# Autodesk Inventor assembly: Omnibot_battery_module.brd
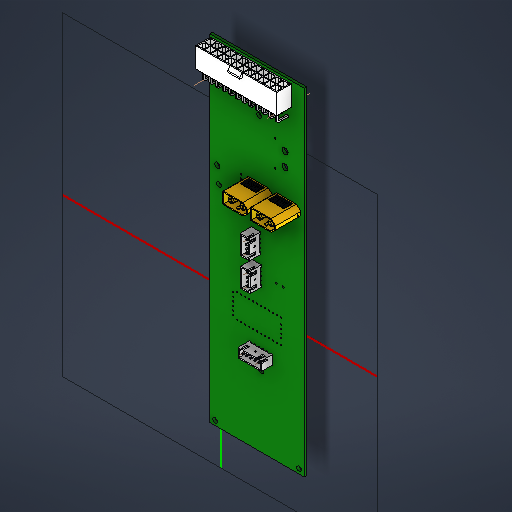
[picture p0: Inventor's stored thumbnail of the model, 512x512]
Saved by Autodesk Inventor 2025 (Build 290162000, 162)
## iProperties
Created: 2024-08-13
Part Number: Omnibot_battery_module.brd
Document SubType Name: Assembly
Designer: IvanPetrov
Author: IvanPetrov
## Documents named in this file (6)
- D:\Projects\OmniBot\design\000.007 - Монитор заряда АКБ.iam
- D:\Projects\OmniBot\design\standart_components\ATX Connector 24pin 90deg\ATX Connector 24pin 90deg.ipt
- D:\Projects\OmniBot\design\standart_components\XT60FemaleConnector.ipt
- D:\Projects\OmniBot\design\standart_components\connectrs\JST - XH - Thru (V) - 4Pin - 2.54mm.ipt
- D:\Projects\OmniBot\design\standart_components\connectrs\JST - XH - Thru (V) - 5Pin - 2.54mm.ipt
- D:\Projects\OmniBot\design\000.007.001 - Плата.ipt
## Components (7 placed, 5 different names)
1. 000.007.001 - Плата:3
2. ATX Connector 24pin 90deg:1 — Угол:5
3. XT60FemaleConnector:1 — Угол:3, Угол:5, Угол:6
4. XT60FemaleConnector:2 — Угол:3, Угол:6
5. JST - XH - Thru (V) - 4Pin - 2.54mm:1
6. JST - XH - Thru (V) - 4Pin - 2.54mm:2
7. JST - XH - Thru (V) - 5Pin - 2.54mm:1
## Relationships (19: Mate 15, Angle 4)
- Угол:3 [Angle] (0 deg): XT60FemaleConnector:1 ↔ XT60FemaleConnector:2
- [Mate]: 000.007.001 - Плата:3 ↔ ATX Connector 24pin 90deg:1
- [Mate]: 000.007.001 - Плата:3 ↔ ATX Connector 24pin 90deg:1
- [Angle] (0 deg): 000.007.001 - Плата:3 ↔ ATX Connector 24pin 90deg:1
- [Mate]: 000.007.001 - Плата:3 ↔ XT60FemaleConnector:1
- [Mate]: 000.007.001 - Плата:3 ↔ XT60FemaleConnector:1
- Угол:5 [Angle] (180 deg): ATX Connector 24pin 90deg:1 ↔ XT60FemaleConnector:1
- [Mate]: 000.007.001 - Плата:3 ↔ XT60FemaleConnector:2
- [Mate]: 000.007.001 - Плата:3 ↔ XT60FemaleConnector:2
- Угол:6 [Angle] (0 deg): XT60FemaleConnector:1 ↔ XT60FemaleConnector:2
- [Mate]: 000.007.001 - Плата:3 ↔ JST - XH - Thru (V) - 5Pin - 2.54mm:1
- [Mate]: 000.007.001 - Плата:3 ↔ JST - XH - Thru (V) - 5Pin - 2.54mm:1
- [Mate]: 000.007.001 - Плата:3 ↔ JST - XH - Thru (V) - 5Pin - 2.54mm:1
- [Mate]: 000.007.001 - Плата:3 ↔ JST - XH - Thru (V) - 4Pin - 2.54mm:2
- [Mate]: 000.007.001 - Плата:3 ↔ JST - XH - Thru (V) - 4Pin - 2.54mm:2
- [Mate]: 000.007.001 - Плата:3 ↔ JST - XH - Thru (V) - 4Pin - 2.54mm:2
- [Mate]: 000.007.001 - Плата:3 ↔ JST - XH - Thru (V) - 4Pin - 2.54mm:1
- [Mate]: 000.007.001 - Плата:3 ↔ JST - XH - Thru (V) - 4Pin - 2.54mm:1
- [Mate]: 000.007.001 - Плата:3 ↔ JST - XH - Thru (V) - 4Pin - 2.54mm:1
